# Autodesk Inventor assembly: Intake
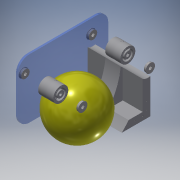
[picture p0: Inventor's stored thumbnail of the model, 180x180]
Saved by Autodesk Inventor 2019 (Build 230136000, 136)
## iProperties
Created: 2020-01-13
Part Number: Intake
Document SubType Name: Assembly
Designer: james
Author: james
## Documents named in this file (6)
- F:\JimsRobot\FIRSTRobots\Design\JimsCHS2020FRC\Intake.iam
- F:\JimsRobot\FIRSTRobots\Design\JimsCHS2020FRC\BottomRamp.ipt
- F:\JimsRobot\FIRSTRobots\Design\JimsCHS2020FRC\BottomRampPlate.ipt
- F:\JimsRobot\FIRSTRobots\Design\Library\AndyMark\am-0692 FR6ZZL-hex.ipt
- F:\JimsRobot\FIRSTRobots\Design\Library\AndyMark\am-3436 2IN 375Hex Stealth Wheel REV2.iam
- F:\JimsRobot\FIRSTRobots\Design\JimsCHS2020FRC\Ball.ipt
## Components (12 placed, 5 different names)
1. BottomRamp:1 — Mate:1, Mate:2, Mate:3, Mate:4, Mate:5, Mate:6
2. BottomRampPlate:1 — Mate:2, Mate:3, Mate:4, Mate:7, Mate:8, Mate:13, Mate:14
3. BottomRampPlate:2 — Mate:1, Mate:5, Mate:6, Mate:9, Mate:10, Mate:11, Mate:12
4. am-0692 FR6ZZL-hex:1 — Mate:10, Mate:12, Mate:17
5. am-0692 FR6ZZL-hex:2 — Mate:7, Mate:13
6. am-0692 FR6ZZL-hex:3 — Mate:8, Mate:14
7. am-0692 FR6ZZL-hex:4 — Mate:9, Mate:11, Mate:20
8. am-3436 2IN 375Hex Stealth Wheel REV2:1 [sub-assembly] — Mate:15, Mate:16, Mate:17
9. am-3436 2IN 375Hex Stealth Wheel REV2:2 [sub-assembly] — Mate:15, Mate:16
10. am-3436 2IN 375Hex Stealth Wheel REV2:3 [sub-assembly] — Mate:18, Mate:19
11. am-3436 2IN 375Hex Stealth Wheel REV2:4 [sub-assembly] — Mate:18, Mate:19, Mate:20
12. Ball:1
## Relationships (20: Mate 20)
- Mate:1: BottomRamp:1 ↔ BottomRampPlate:2
- Mate:2: BottomRamp:1 ↔ BottomRampPlate:1
- Mate:3: BottomRamp:1 ↔ BottomRampPlate:1
- Mate:4: BottomRamp:1 ↔ BottomRampPlate:1
- Mate:5: BottomRamp:1 ↔ BottomRampPlate:2
- Mate:6: BottomRamp:1 ↔ BottomRampPlate:2
- Mate:7: BottomRampPlate:1 ↔ am-0692 FR6ZZL-hex:2
- Mate:8: BottomRampPlate:1 ↔ am-0692 FR6ZZL-hex:3
- Mate:9: BottomRampPlate:2 ↔ am-0692 FR6ZZL-hex:4
- Mate:10: BottomRampPlate:2 ↔ am-0692 FR6ZZL-hex:1
- Mate:11: BottomRampPlate:2 ↔ am-0692 FR6ZZL-hex:4
- Mate:12: BottomRampPlate:2 ↔ am-0692 FR6ZZL-hex:1
- Mate:13: BottomRampPlate:1 ↔ am-0692 FR6ZZL-hex:2
- Mate:14: BottomRampPlate:1 ↔ am-0692 FR6ZZL-hex:3
- Mate:15: am-3436 2IN 375Hex Stealth Wheel REV2:1 ↔ am-3436 2IN 375Hex Stealth Wheel REV2:2
- Mate:16: am-3436 2IN 375Hex Stealth Wheel REV2:1 ↔ am-3436 2IN 375Hex Stealth Wheel REV2:2
- Mate:17: am-0692 FR6ZZL-hex:1 ↔ am-3436 2IN 375Hex Stealth Wheel REV2:1
- Mate:18: am-3436 2IN 375Hex Stealth Wheel REV2:3 ↔ am-3436 2IN 375Hex Stealth Wheel REV2:4
- Mate:19: am-3436 2IN 375Hex Stealth Wheel REV2:3 ↔ am-3436 2IN 375Hex Stealth Wheel REV2:4
- Mate:20: am-0692 FR6ZZL-hex:4 ↔ am-3436 2IN 375Hex Stealth Wheel REV2:4
